# Autodesk Inventor assembly: GabelBottom_Link_COG
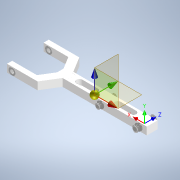
[picture p0: Inventor's stored thumbnail of the model, 180x180]
Saved by Autodesk Inventor 2022 (Build 260153000, 153)
## iProperties
Created: 2022-10-18
Part Number: GabelBottom_Link_COG
Document SubType Name: Assembly
Designer: alexw
Mass: 305.825 g
Surface Area: 588.56 cm^2
Volume: 185.62 cm^3
Density: 1.64758 g/cm^3
Author: alexw
## Documents named in this file (4)
- C:\Users\alexw\Documents\Inventor\Projects\03_CurrentProjects\MasterThesis\PSM_V1_Rillenkugellager\COG\GabelBottom_Link_COG.iam
- C:\Users\alexw\Documents\Inventor\Projects\03_CurrentProjects\MasterThesis\PSM_V1_Rillenkugellager\Adaptationhorizontalachse_Assembly_Rillenkugellager.iam
- C:\Users\alexw\Documents\Inventor\Projects\03_CurrentProjects\MasterThesis\PSM_V1_Rillenkugellager\Maschinenbauteil\circlips_din471_8_0_8.ipt
- C:\Users\alexw\Documents\Inventor\Projects\03_CurrentProjects\MasterThesis\PSM_V1_Rillenkugellager\Maschinenbauteil\din_988_8_x_14_x_0_10.ipt
## Components (5 placed, 3 different names)
1. Adaptationhorizontalachse_Assembly_Rillenkugellager:1 [sub-assembly] — Passend:1, Passend:2, Passend:3, Passend:4, Passend:5, Passend:7, Passend:9, Passend:10, Winkel:1, Passend:11
2. circlips_din471_8_0_8:1 — Passend:5, Passend:6
3. circlips_din471_8_0_8:2 — Passend:7, Passend:8
4. din_988_8_x_14_x_0_10:1 — Passend:1, Passend:2, Passend:6
5. din_988_8_x_14_x_0_10:2 — Passend:3, Passend:4, Passend:8
## Relationships (12: Mate 11, Angle 1)
- Passend:1 [Mate]: Adaptationhorizontalachse_Assembly_Rillenkugellager:1 ↔ din_988_8_x_14_x_0_10:1
- Passend:2 [Mate]: Adaptationhorizontalachse_Assembly_Rillenkugellager:1 ↔ din_988_8_x_14_x_0_10:1
- Passend:3 [Mate]: Adaptationhorizontalachse_Assembly_Rillenkugellager:1 ↔ din_988_8_x_14_x_0_10:2
- Passend:4 [Mate]: Adaptationhorizontalachse_Assembly_Rillenkugellager:1 ↔ din_988_8_x_14_x_0_10:2
- Passend:5 [Mate]: Adaptationhorizontalachse_Assembly_Rillenkugellager:1 ↔ circlips_din471_8_0_8:1
- Passend:6 [Mate]: circlips_din471_8_0_8:1 ↔ din_988_8_x_14_x_0_10:1
- Passend:7 [Mate]: Adaptationhorizontalachse_Assembly_Rillenkugellager:1 ↔ circlips_din471_8_0_8:2
- Passend:8 [Mate]: circlips_din471_8_0_8:2 ↔ din_988_8_x_14_x_0_10:2
- Passend:9 [Mate]: Adaptationhorizontalachse_Assembly_Rillenkugellager:1
- Passend:10 [Mate]: Adaptationhorizontalachse_Assembly_Rillenkugellager:1
- Winkel:1 [Angle] (0 deg): Adaptationhorizontalachse_Assembly_Rillenkugellager:1
- Passend:11 [Mate]: Adaptationhorizontalachse_Assembly_Rillenkugellager:1
